# Autodesk Inventor assembly: Assembly
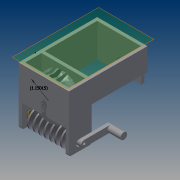
[picture p0: Inventor's stored thumbnail of the model, 180x180]
Saved by Autodesk Inventor 2015 SP1 (Build 190203100, 203)
## iProperties
Created: 2015-04-25
Part Number: Assembly
Document SubType Name: Assembly
Designer: Trevor
Author: Trevor
## Documents named in this file (5)
- C:\Users\Trevor\Google Drive\Classwork\6.S079\Project\6.s079-musicbox\CAD\Assembly.iam
- C:\Users\Trevor\Google Drive\Classwork\6.S079\Project\6.s079-musicbox\CAD\Assembly\Design Accelerator\Worm Gears1.iam
- C:\Users\Trevor\Google Drive\Classwork\6.S079\Project\6.s079-musicbox\CAD\Assembly\Design Accelerator\Worm1.ipt
- C:\Users\Trevor\Google Drive\Classwork\6.S079\Project\6.s079-musicbox\CAD\Crank.ipt
- C:\Users\Trevor\Google Drive\Classwork\6.S079\Project\6.s079-musicbox\CAD\Box.ipt
## Components (3 placed, 3 different names)
1. Worm Gears:1 [sub-assembly] — Mate:1, Mate:2, Rotation:1, Mate:3
2. Crank:1 — Mate:1, Mate:2, Rotation:1, Mate:3
3. Box:1 — Flush:1
## Relationships (5: Mate 3, RelateRotation 1, Flush 1)
- Mate:1: Worm Gears:1 ↔ Crank:1
- Mate:2: Worm Gears:1 ↔ Crank:1
- Rotation:1 [RelateRotation] (0.312 ul): Worm Gears:1 ↔ Crank:1
- Mate:3: Worm Gears:1 ↔ Crank:1
- Flush:1: Box:1
## Named parameters: l_key = 6.73519 mm, d_key = 6.35 mm
